# Autodesk Inventor assembly: MPPC Sensor V4 Populated
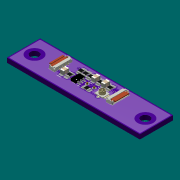
[picture p0: Inventor's stored thumbnail of the model, 180x180]
Saved by Autodesk Inventor 2016 (Build 200138000, 138)
## iProperties
Created: 2015-08-26
Part Number: MPPC Sensor V4 Populated
Document SubType Name: Assembly
Designer: Cosmic
Author: Cosmic
## Documents named in this file (8)
- C:\Users\Sawaiz\Documents\pcb\mppcSensorInterface\cad\sensor.iam
- C:\Users\Sawaiz\Documents\pcb\mppcSensorInterface\cad\pcb.ipt
- C:\Users\Sawaiz\Documents\pcb\mppcSensorInterface\cad\electronics\0805.ipt
- C:\Users\Sawaiz\Documents\pcb\mppcSensorInterface\cad\electronics\0805 Capacitor.ipt
- C:\Users\Sawaiz\Documents\pcb\mppcSensorInterface\cad\electronics\128-0711-201.ipt
- C:\Users\Sawaiz\Documents\pcb\mppcSensorInterface\cad\electronics\SOT23_5.ipt
- C:\Users\Sawaiz\Documents\pcb\mppcSensorInterface\cad\electronics\FH33-4S-1SH.ipt
- C:\Users\Sawaiz\Documents\pcb\mppcSensorInterface\cad\electronics\MPPC.ipt
## Components (16 placed, 7 different names)
1. pcb:1 — Angle:1, Angle:2, Angle:3, Mate:1, Angle:5, Mate:2, Angle:6, Mate:3, Angle:7, Mate:4, Mate:5, Mate:6, Angle:8, Angle:9, Mate:7, Mate:8, Mate:9
2. 0805:1 — Flush:5, Flush:8, Flush:9
3. 0805:2 — Flush:4, Flush:5, Flush:7, Flush:8
4. 0805:3 — Flush:3, Flush:4, Flush:6, Flush:7
5. 0805:4 — Flush:2, Flush:3, Flush:6
6. 0805:5 — Flush:1, Flush:9, Angle:1, Flush:10
7. 0805:6 — Flush:1, Flush:2, Angle:3, Mate:1
8. 0805:7 — Flush:10, Angle:2
9. 0805 Capacitor:1 — Flush:11, Flush:12, Angle:4, Angle:5, Flush:13
10. 0805 Capacitor:2 — Flush:11, Flush:13
11. 0805 Capacitor:3 — Flush:12, Angle:4, Mate:2
12. 128-0711-201:1 — Angle:6, Mate:3
13. SOT23_5:1 — Angle:7, Mate:4
14. FH33-4S-1SH:1 — Mate:6, Angle:9
15. FH33-4S-1SH:2 — Mate:5, Angle:8
16. MPPC:1 — Mate:7, Mate:8, Mate:9
## Relationships (31: Flush 13, Angle 9, Mate 9)
- Flush:1: 0805:5 ↔ 0805:6
- Flush:2: 0805:4 ↔ 0805:6
- Flush:3: 0805:3 ↔ 0805:4
- Flush:4: 0805:2 ↔ 0805:3
- Flush:5: 0805:1 ↔ 0805:2
- Flush:6: 0805:3 ↔ 0805:4
- Flush:7: 0805:2 ↔ 0805:3
- Flush:8: 0805:1 ↔ 0805:2
- Flush:9: 0805:1 ↔ 0805:5
- Angle:1 (0 deg): pcb:1 ↔ 0805:5
- Flush:10: 0805:5 ↔ 0805:7
- Angle:2 (0 deg): pcb:1 ↔ 0805:7
- Angle:3 (0 deg): pcb:1 ↔ 0805:6
- Mate:1: pcb:1 ↔ 0805:6
- Flush:11: 0805 Capacitor:1 ↔ 0805 Capacitor:2
- Flush:12: 0805 Capacitor:1 ↔ 0805 Capacitor:3
- Angle:4 (0 deg): 0805 Capacitor:1 ↔ 0805 Capacitor:3
- Angle:5 (0 deg): pcb:1 ↔ 0805 Capacitor:1
- Flush:13: 0805 Capacitor:1 ↔ 0805 Capacitor:2
- Mate:2: pcb:1 ↔ 0805 Capacitor:3
- Angle:6 (0 deg): pcb:1 ↔ 128-0711-201:1
- Mate:3: pcb:1 ↔ 128-0711-201:1
- Angle:7 (0 deg): pcb:1 ↔ SOT23_5:1
- Mate:4: pcb:1 ↔ SOT23_5:1
- Mate:5: pcb:1 ↔ FH33-4S-1SH:2
- Mate:6: pcb:1 ↔ FH33-4S-1SH:1
- Angle:8 (0 deg): pcb:1 ↔ FH33-4S-1SH:2
- Angle:9 (0 deg): pcb:1 ↔ FH33-4S-1SH:1
- Mate:7: pcb:1 ↔ MPPC:1
- Mate:8: pcb:1 ↔ MPPC:1
- Mate:9: pcb:1 ↔ MPPC:1
